# Autodesk Inventor assembly: GCS_Ax2
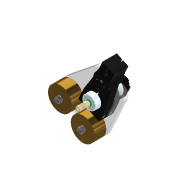
[picture p0: Inventor's stored thumbnail of the model, 180x180]
Saved by Autodesk Inventor 2022 (Build 260153000, 153)
## iProperties
Created: 2022-12-23
Part Number: GCS_Ax2
Document SubType Name: Assembly
Designer: alexw
Author: alexw
## Documents named in this file (4)
- C:\Users\alexw\Documents\Inventor\Projects\03_CurrentProjects\MasterThesis\PSM_V1_Rillenkugellager\GCS_Ax2.iam
- C:\Users\alexw\Documents\Inventor\Projects\03_CurrentProjects\MasterThesis\PSM_V1_Rillenkugellager\MorotFixation_CounterWeightHolder_Assembly.iam
- C:\Users\alexw\Documents\Inventor\Projects\03_CurrentProjects\MasterThesis\PSM_V1_Rillenkugellager\DMP_counterweight_Assembly.iam
- C:\Users\alexw\Documents\Inventor\Projects\03_CurrentProjects\MasterThesis\PSM_V1_Rillenkugellager\ContentCenter\de-DE\ISO 4762(2)\ISO 4762 - M4 x 30ISO.ipt
## Components (3 placed, 3 different names)
1. MorotFixation_CounterWeightHolder_Assembly:1 [sub-assembly]
2. DMP_counterweight_Assembly:1 [sub-assembly]
3. ISO 4762 M4 x 30:1
## Relationships (5: Mate 5)
- [Mate]: MorotFixation_CounterWeightHolder_Assembly:1 ↔ DMP_counterweight_Assembly:1
- [Mate]: MorotFixation_CounterWeightHolder_Assembly:1 ↔ DMP_counterweight_Assembly:1
- [Mate]: MorotFixation_CounterWeightHolder_Assembly:1 ↔ DMP_counterweight_Assembly:1
- [Mate]: DMP_counterweight_Assembly:1 ↔ ISO 4762 M4 x 30:1
- [Mate]: DMP_counterweight_Assembly:1 ↔ ISO 4762 M4 x 30:1
